# Autodesk Inventor assembly: SecuroBot Assembly
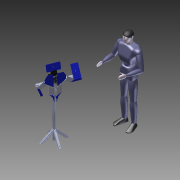
[picture p0: Inventor's stored thumbnail of the model, 180x180]
Saved by Autodesk Inventor 2014 SP2 (Build 180246200, 246)
## iProperties
Created: 2015-07-31
Part Number: SecuroBot Assembly
Document SubType Name: Assembly
Designer: Devon
Author: Devon
## Documents named in this file (31)
- C:\Users\Devon\Downloads\SecuroBot_Hardware_Files-2015-10-11\SecuroBot Hardware Files\CAD Files\SecuroBot Assembly.iam
- C:\Users\Devon\Downloads\SecuroBot_Hardware_Files-2015-10-11\SecuroBot Hardware Files\CAD Files\Milled Extrusion Parts\Leg.ipt
- C:\Users\Devon\Downloads\SecuroBot_Hardware_Files-2015-10-11\SecuroBot Hardware Files\CAD Files\Milled Extrusion Parts\Spine.ipt
- C:\Users\Devon\Downloads\SecuroBot_Hardware_Files-2015-10-11\SecuroBot Hardware Files\CAD Files\Milled Extrusion Parts\Left Arm.ipt
- C:\Users\Devon\Downloads\SecuroBot_Hardware_Files-2015-10-11\SecuroBot Hardware Files\CAD Files\3D Printed Parts\Rotating Base mount.ipt
- C:\Users\Devon\Downloads\SecuroBot_Hardware_Files-2015-10-11\SecuroBot Hardware Files\CAD Files\Purchased Parts\Rotating Base - simplified model.ipt
- C:\Users\Devon\Downloads\SecuroBot_Hardware_Files-2015-10-11\SecuroBot Hardware Files\CAD Files\Imported Components\ANGLE BRACE\ANGLE BRACE.ipt
- C:\Users\Devon\Downloads\SecuroBot_Hardware_Files-2015-10-11\SecuroBot Hardware Files\CAD Files\Imported Components\person\person.ipt
- C:\Users\Devon\Downloads\SecuroBot_Hardware_Files-2015-10-11\SecuroBot Hardware Files\CAD Files\Imported Components\enclosure\enclosure.ipt
- C:\Users\Devon\Downloads\SecuroBot_Hardware_Files-2015-10-11\SecuroBot Hardware Files\CAD Files\3D Printed Parts\Left Abdomen.ipt
- C:\Users\Devon\Downloads\SecuroBot_Hardware_Files-2015-10-11\SecuroBot Hardware Files\CAD Files\3D Printed Parts\Left Chest.ipt
- C:\Users\Devon\Downloads\SecuroBot_Hardware_Files-2015-10-11\SecuroBot Hardware Files\CAD Files\3D Printed Parts\Left Hip.ipt
- C:\Users\Devon\Downloads\SecuroBot_Hardware_Files-2015-10-11\SecuroBot Hardware Files\CAD Files\3D Printed Parts\Right Abdomen.ipt
- C:\Users\Devon\Downloads\SecuroBot_Hardware_Files-2015-10-11\SecuroBot Hardware Files\CAD Files\3D Printed Parts\Right Chest.ipt
- C:\Users\Devon\Downloads\SecuroBot_Hardware_Files-2015-10-11\SecuroBot Hardware Files\CAD Files\3D Printed Parts\Right Hip.ipt
- C:\Users\Devon\Downloads\SecuroBot_Hardware_Files-2015-10-11\SecuroBot Hardware Files\CAD Files\3D Printed Parts\Left Bicep.ipt
- C:\Users\Devon\Downloads\SecuroBot_Hardware_Files-2015-10-11\SecuroBot Hardware Files\CAD Files\3D Printed Parts\Left Forearm.ipt
- C:\Users\Devon\Downloads\SecuroBot_Hardware_Files-2015-10-11\SecuroBot Hardware Files\CAD Files\3D Printed Parts\Right Bicep.ipt
- C:\Users\Devon\Downloads\SecuroBot_Hardware_Files-2015-10-11\SecuroBot Hardware Files\CAD Files\3D Printed Parts\Right Forearm.ipt
- C:\Users\Devon\Downloads\SecuroBot_Hardware_Files-2015-10-11\SecuroBot Hardware Files\CAD Files\3D Printed Parts\Master Tablet Cover.ipt
- C:\Users\Devon\Downloads\SecuroBot_Hardware_Files-2015-10-11\SecuroBot Hardware Files\CAD Files\3D Printed Parts\Master Tablet Enclosure.ipt
- C:\Users\Devon\Downloads\SecuroBot_Hardware_Files-2015-10-11\SecuroBot Hardware Files\CAD Files\3D Printed Parts\Slave Tablet Cover.ipt
- C:\Users\Devon\Downloads\SecuroBot_Hardware_Files-2015-10-11\SecuroBot Hardware Files\CAD Files\3D Printed Parts\Slave Tablet Enclosure.ipt
- C:\Users\Devon\Downloads\SecuroBot_Hardware_Files-2015-10-11\SecuroBot Hardware Files\CAD Files\Purchased Parts\ANGLE BRACE.ipt
- C:\Users\Devon\Downloads\SecuroBot_Hardware_Files-2015-10-11\SecuroBot Hardware Files\CAD Files\3D Printed Parts\Chest Standoff.ipt
- C:\Users\Devon\Downloads\SecuroBot_Hardware_Files-2015-10-11\SecuroBot Hardware Files\CAD Files\3D Printed Parts\IR Cover.ipt
- C:\Users\Devon\Downloads\SecuroBot_Hardware_Files-2015-10-11\SecuroBot Hardware Files\CAD Files\3D Printed Parts\Master Tablet and IR Mount.ipt
- C:\Users\Devon\Downloads\SecuroBot_Hardware_Files-2015-10-11\SecuroBot Hardware Files\CAD Files\3D Printed Parts\Speaker Front Plate.ipt
- C:\Users\Devon\Downloads\SecuroBot_Hardware_Files-2015-10-11\SecuroBot Hardware Files\CAD Files\Purchased Parts\speaker body.ipt
- C:\Users\Devon\Downloads\SecuroBot_Hardware_Files-2015-10-11\SecuroBot Hardware Files\CAD Files\Milled Extrusion Parts\Right Arm Standoff.ipt
- C:\Users\Devon\Downloads\SecuroBot_Hardware_Files-2015-10-11\SecuroBot Hardware Files\CAD Files\Milled Extrusion Parts\Right Arm.ipt
## Components (39 placed, 29 different names)
1. Leg:1 — Mate:2, Flush:3, Flush:4
2. Spine:1 — Mate:2, Flush:3, Flush:4, Mate:4, Flush:7, Flush:8, Mate:5, Flush:9, Flush:10, Mate:6, Flush:11, Flush:12, Mate:7, Flush:13, Mate:10, Flush:16, Mate:13, Flush:17, Mate:14, Flush:18, Mate:16, Flush:19, Insert:1, Mate:42, Mate:43, Flush:31, Flush:32, Mate:47, Flush:33, Mate:49, Flush:34, Mate:51, Mate:52, Flush:35, Flush:36, Mate:78, Flush:51, Mate:79, Mate:80, Mate:88, Mate:91, Flush:57
3. Leg:2 — Mate:4, Flush:7, Flush:8, Flush:27
4. Leg:3 — Mate:5, Flush:9, Flush:10
5. Leg:4 — Mate:6, Flush:11, Flush:12
6. Left Arm:1 — Mate:7, Flush:13, Mate:55, Flush:37, Mate:57, Flush:38, Mate:76, Mate:77, Mate:86, Flush:56, Flush:58
7. Rotating Base mount:1 — Mate:9, Flush:14, Flush:15, Mate:11, Mate:12, Mate:15, Mate:17, Insert:1
8. Rotating Base - simplified model:1 — Mate:9, Flush:14, Flush:15, Flush:29, Flush:30, Mate:81, Insert:4
9. ANGLE BRACE:1 — Mate:14, Mate:15, Flush:18, Mate:44
10. ANGLE BRACE:2 — Mate:12, Mate:13, Flush:17
11. ANGLE BRACE:3 — Mate:10, Mate:11, Flush:16, Mate:89
12. ANGLE BRACE:4 — Mate:16, Mate:17, Flush:19
13. person:1 — Flush:27
14. enclosure:1 — Mate:42, Mate:43, Mate:44, Mate:87
15. Left Abdomen:1 — Mate:47, Flush:33, Mate:48, Mate:53
16. Left Chest:1 — Flush:29, Flush:31, Mate:48, Mate:56, Mate:66, Insert:2, Mate:90
17. Left Hip:1 — Mate:51, Flush:36, Mate:53
18. Right Abdomen:1 — Mate:49, Flush:34, Mate:50, Mate:54
19. Right Chest:1 — Flush:30, Flush:32, Mate:50, Mate:59, Mate:60, Flush:39, Insert:3
20. Right Hip:1 — Mate:52, Flush:35, Mate:54
21. Left Bicep:1 — Mate:55, Mate:56, Flush:37, Mate:58, Mate:66
22. Left Forearm:1 — Mate:57, Flush:38, Mate:58, Mate:75, Flush:50
23. Right Bicep:1 — Mate:59, Mate:60, Flush:39, Flush:40, Mate:61, Flush:41
24. Right Forearm:1 — Flush:40, Mate:61, Flush:41
25. Master Tablet Cover:1 — Mate:65, Flush:44, Flush:45
26. Master Tablet Enclosure:1 — Mate:65, Flush:44, Flush:45, Mate:83, Insert:6, Insert:7
27. Slave Tablet Cover:1 — Mate:71, Flush:48, Flush:49
28. Slave Tablet Enclosure:1 — Mate:71, Flush:48, Flush:49, Mate:75, Mate:76, Flush:50
29. ANGLE BRACE:1 — Mate:77, Mate:78, Flush:51
30. Chest Standoff:1 — Mate:79, Insert:2
31. Chest Standoff:2 — Mate:80, Insert:3
32. IR Cover:1 — Mate:82, Insert:5
33. Master Tablet and IR Mount:1 — Mate:81, Insert:4, Mate:82, Insert:5, Mate:83, Insert:6, Insert:7
34. Speaker Front Plate:1 — Mate:84, Flush:52, Flush:53
35. Speaker Front Plate:2 — Mate:85, Flush:54, Flush:55, Flush:56
36. speaker body:1 — Mate:84, Flush:52, Flush:53, Mate:88, Mate:89, Mate:90
37. speaker body:2 — Mate:85, Flush:54, Flush:55, Mate:86, Mate:87
38. Right Arm Standoff:1 — Mate:92, Flush:59, Flush:60
39. Right Arm:1 — Mate:91, Flush:57, Flush:58, Mate:92, Flush:59, Flush:60
## Relationships (104: Mate 53, Flush 44, Insert 7)
- Mate:2: Leg:1 ↔ Spine:1
- Flush:3: Leg:1 ↔ Spine:1
- Flush:4: Leg:1 ↔ Spine:1
- Mate:4: Spine:1 ↔ Leg:2
- Flush:7: Spine:1 ↔ Leg:2
- Flush:8: Spine:1 ↔ Leg:2
- Mate:5: Spine:1 ↔ Leg:3
- Flush:9: Spine:1 ↔ Leg:3
- Flush:10: Spine:1 ↔ Leg:3
- Mate:6: Spine:1 ↔ Leg:4
- Flush:11: Spine:1 ↔ Leg:4
- Flush:12: Spine:1 ↔ Leg:4
- Mate:7: Spine:1 ↔ Left Arm:1
- Flush:13: Spine:1 ↔ Left Arm:1
- Mate:9: Rotating Base mount:1 ↔ Rotating Base - simplified model:1
- Flush:14: Rotating Base mount:1 ↔ Rotating Base - simplified model:1
- Flush:15: Rotating Base mount:1 ↔ Rotating Base - simplified model:1
- Mate:10: Spine:1 ↔ ANGLE BRACE:3
- Mate:11: Rotating Base mount:1 ↔ ANGLE BRACE:3
- Flush:16: Spine:1 ↔ ANGLE BRACE:3
- Mate:12: Rotating Base mount:1 ↔ ANGLE BRACE:2
- Mate:13: Spine:1 ↔ ANGLE BRACE:2
- Flush:17: Spine:1 ↔ ANGLE BRACE:2
- Mate:14: Spine:1 ↔ ANGLE BRACE:1
- Mate:15: Rotating Base mount:1 ↔ ANGLE BRACE:1
- Flush:18: Spine:1 ↔ ANGLE BRACE:1
- Mate:16: Spine:1 ↔ ANGLE BRACE:4
- Mate:17: Rotating Base mount:1 ↔ ANGLE BRACE:4
- Flush:19: Spine:1 ↔ ANGLE BRACE:4
- Insert:1: Spine:1 ↔ Rotating Base mount:1
- Flush:27: Leg:2 ↔ person:1
- Mate:42: Spine:1 ↔ enclosure:1
- Mate:43 (31.75 mm): Spine:1 ↔ enclosure:1
- Mate:44 (76.2 mm): ANGLE BRACE:1 ↔ enclosure:1
- Flush:29: Rotating Base - simplified model:1 ↔ Left Chest:1
- Flush:30: Rotating Base - simplified model:1 ↔ Right Chest:1
- Flush:31: Spine:1 ↔ Left Chest:1
- Flush:32: Spine:1 ↔ Right Chest:1
- Mate:47: Spine:1 ↔ Left Abdomen:1
- Flush:33: Spine:1 ↔ Left Abdomen:1
- Mate:48 (12.7 mm): Left Abdomen:1 ↔ Left Chest:1
- Mate:49: Spine:1 ↔ Right Abdomen:1
- Flush:34: Spine:1 ↔ Right Abdomen:1
- Mate:50 (12.7 mm): Right Abdomen:1 ↔ Right Chest:1
- Mate:51: Spine:1 ↔ Left Hip:1
- Mate:52: Spine:1 ↔ Right Hip:1
- Flush:35: Spine:1 ↔ Right Hip:1
- Flush:36: Spine:1 ↔ Left Hip:1
- Mate:53 (12.7 mm): Left Abdomen:1 ↔ Left Hip:1
- Mate:54 (12.7 mm): Right Abdomen:1 ↔ Right Hip:1
- Mate:55: Left Arm:1 ↔ Left Bicep:1
- Mate:56 (12.7 mm): Left Chest:1 ↔ Left Bicep:1
- Flush:37: Left Arm:1 ↔ Left Bicep:1
- Mate:57: Left Arm:1 ↔ Left Forearm:1
- Flush:38: Left Arm:1 ↔ Left Forearm:1
- Mate:58 (12.7 mm): Left Bicep:1 ↔ Left Forearm:1
- Mate:59: Right Chest:1 ↔ Right Bicep:1
- Mate:60: Right Chest:1 ↔ Right Bicep:1
- Flush:39: Right Chest:1 ↔ Right Bicep:1
- Flush:40: Right Bicep:1 ↔ Right Forearm:1
- Mate:61: Right Bicep:1 ↔ Right Forearm:1
- Flush:41: Right Bicep:1 ↔ Right Forearm:1
- Mate:65: Master Tablet Cover:1 ↔ Master Tablet Enclosure:1
- Flush:44: Master Tablet Cover:1 ↔ Master Tablet Enclosure:1
- Flush:45: Master Tablet Cover:1 ↔ Master Tablet Enclosure:1
- Mate:66 (12.7 mm): Left Chest:1 ↔ Left Bicep:1
- Mate:71: Slave Tablet Cover:1 ↔ Slave Tablet Enclosure:1
- Flush:48: Slave Tablet Cover:1 ↔ Slave Tablet Enclosure:1
- Flush:49: Slave Tablet Cover:1 ↔ Slave Tablet Enclosure:1
- Mate:75: Left Forearm:1 ↔ Slave Tablet Enclosure:1
- Mate:76: Left Arm:1 ↔ Slave Tablet Enclosure:1
- Flush:50: Left Forearm:1 ↔ Slave Tablet Enclosure:1
- Mate:77: Left Arm:1 ↔ ANGLE BRACE:1
- Mate:78: Spine:1 ↔ ANGLE BRACE:1
- Flush:51: Spine:1 ↔ ANGLE BRACE:1
- Mate:79: Spine:1 ↔ Chest Standoff:1
- Mate:80: Spine:1 ↔ Chest Standoff:2
- Insert:2: Left Chest:1 ↔ Chest Standoff:1
- Insert:3: Right Chest:1 ↔ Chest Standoff:2
- Mate:81: Rotating Base - simplified model:1 ↔ Master Tablet and IR Mount:1
- Insert:4: Rotating Base - simplified model:1 ↔ Master Tablet and IR Mount:1
- Mate:82: IR Cover:1 ↔ Master Tablet and IR Mount:1
- Insert:5: IR Cover:1 ↔ Master Tablet and IR Mount:1
- Mate:83: Master Tablet Enclosure:1 ↔ Master Tablet and IR Mount:1
- Insert:6: Master Tablet Enclosure:1 ↔ Master Tablet and IR Mount:1
- Insert:7: Master Tablet Enclosure:1 ↔ Master Tablet and IR Mount:1
- Mate:84: Speaker Front Plate:1 ↔ speaker body:1
- Flush:52: Speaker Front Plate:1 ↔ speaker body:1
- Flush:53: Speaker Front Plate:1 ↔ speaker body:1
- Mate:85: Speaker Front Plate:2 ↔ speaker body:2
- Flush:54: Speaker Front Plate:2 ↔ speaker body:2
- Flush:55: Speaker Front Plate:2 ↔ speaker body:2
- Mate:86: Left Arm:1 ↔ speaker body:2
- Flush:56: Left Arm:1 ↔ Speaker Front Plate:2
- Mate:87 (25.4 mm): enclosure:1 ↔ speaker body:2
- Mate:88: Spine:1 ↔ speaker body:1
- Mate:89 (12.7 mm): ANGLE BRACE:3 ↔ speaker body:1
- Mate:90 (1.2065 mm): Left Chest:1 ↔ speaker body:1
- Mate:91: Spine:1 ↔ Right Arm:1
- Flush:57: Spine:1 ↔ Right Arm:1
- Flush:58: Left Arm:1 ↔ Right Arm:1
- Mate:92: Right Arm Standoff:1 ↔ Right Arm:1
- Flush:59: Right Arm Standoff:1 ↔ Right Arm:1
- Flush:60 (44.45 mm): Right Arm Standoff:1 ↔ Right Arm:1
